# Autodesk Inventor assembly: Final Assembly
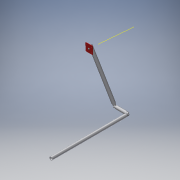
[picture p0: Inventor's stored thumbnail of the model, 180x180]
Saved by Autodesk Inventor 2018 (Build 220112000, 112)
## iProperties
Created: 2018-05-07
Part Number: Final Assembly
Document SubType Name: Assembly
Designer: 232963
Author: 232963
## Documents named in this file (9)
- P:\IED\SchoolCAD\Design Challenge\Final Assembly.iam
- P:\IED\SchoolCAD\Design Challenge\Main Rod.ipt
- P:\IED\SchoolCAD\Design Challenge\Short ROd.ipt
- P:\IED\SchoolCAD\Design Challenge\Slanted rod.ipt
- P:\IED\SchoolCAD\Design Challenge\real joint assemly.iam
- P:\IED\SchoolCAD\Design Challenge\Real Joint assembly 57d.iam
- P:\IED\SchoolCAD\Design Challenge\back plate.ipt
- P:\IED\SchoolCAD\Design Challenge\Bolt.ipt
- P:\IED\SchoolCAD\Design Challenge\Nut.ipt
## Components (8 placed, 8 different names)
1. Main Rod:1 — Insert:1
2. Short ROd:1 — Insert:2, Insert:3
3. real joint assemly:1 [sub-assembly] — Insert:1, Insert:2
4. Real Joint assembly 57d:1 [sub-assembly] — Insert:3, Insert:4
5. back plate:1 — Insert:6
6. Slanted rod:1 — Insert:4, Mate:1, Tangent:1
7. Bolt:1 — Mate:2, Insert:5, Insert:6
8. Nut:1 — Insert:5, Tangent:1
## Relationships (9: Insert 6, Mate 2, Tangent 1)
- Insert:1 (-12.7 mm): Main Rod:1 ↔ real joint assemly:1
- Insert:2 (-12.7 mm): Short ROd:1 ↔ real joint assemly:1
- Insert:3 (-12.7 mm): Short ROd:1 ↔ Real Joint assembly 57d:1
- Insert:4 (-12.7 mm): Real Joint assembly 57d:1 ↔ Slanted rod:1
- Mate:1: Slanted rod:1
- Mate:2: Bolt:1
- Insert:5: Bolt:1 ↔ Nut:1
- Tangent:1: Slanted rod:1 ↔ Nut:1
- Insert:6: back plate:1 ↔ Bolt:1
